# Autodesk Inventor assembly: Custom_Delta_Assembly
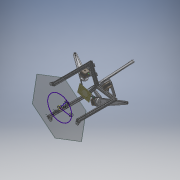
[picture p0: Inventor's stored thumbnail of the model, 180x180]
Saved by Autodesk Inventor 2019 (Build 230136000, 136)
## iProperties
Created: 2019-07-06
Part Number: Custom_Delta_Assembly
Document SubType Name: Assembly
Designer: Jorian Brusind
Author: Jorian Brusind
## Documents named in this file (15)
- C:\Users\Jorian Brusind\Documents\GitHub\ECE44x_Senior_Design\Design files\Delta Robot Arm\Inventor Files\Custom_Delta\Custom_Delta_Assembly.iam
- C:\Users\Jorian Brusind\Documents\GitHub\ECE44x_Senior_Design\Design files\Delta Robot Arm\Inventor Files\Custom_Delta\Stepper_Face.ipt
- C:\Users\Jorian Brusind\Documents\GitHub\ECE44x_Senior_Design\Design files\Delta Robot Arm\Inventor Files\nema-17-stepper-motor-with-v2-damper-1.snapshot.3\Nema 17  Stepper Motor length 34mm.ipt
- C:\Users\Jorian Brusind\Documents\GitHub\ECE44x_Senior_Design\Design files\Delta Robot Arm\Inventor Files\Stepper_Collar\products\12488\step\model.ipt
- C:\Users\Jorian Brusind\Documents\GitHub\ECE44x_Senior_Design\Design files\Delta Robot Arm\Inventor Files\Custom_Delta\Delta_Arm.ipt
- C:\Users\Jorian Brusind\Documents\GitHub\ECE44x_Senior_Design\Design files\Delta Robot Arm\Inventor Files\Custom_Delta\Delta_Top.ipt
- C:\Users\Jorian Brusind\Documents\GitHub\ECE44x_Senior_Design\Design files\Delta Robot Arm\Inventor Files\McMaster Files\59935K140_METRIC BALL JOINT ROD END.ipt
- C:\Users\Jorian Brusind\Documents\GitHub\ECE44x_Senior_Design\Design files\PetriFilm\PetriFilm.iam
- C:\Users\Jorian Brusind\Documents\GitHub\ECE44x_Senior_Design\Design files\Delta Robot Arm\Inventor Files\McMaster Files\5537T501_ALUMINUM T-SLOTTED FRAMING EXTRUSION.ipt
- C:\Users\Jorian Brusind\Documents\GitHub\ECE44x_Senior_Design\Design files\Delta Robot Arm\Inventor Files\McMaster Files\5537T518_T-SLOTTED FRAMING.ipt
- C:\Users\Jorian Brusind\Documents\GitHub\ECE44x_Senior_Design\Design files\Delta Robot Arm\Inventor Files\McMaster Files\6In_ALUMINUM T-SLOTTED FRAMING EXTRUSION.ipt
- C:\Users\Jorian Brusind\Documents\GitHub\ECE44x_Senior_Design\Design files\Delta Robot Arm\Inventor Files\McMaster Files\98861A050_LOW-STRENGTH STEEL THREADED ROD.ipt
- C:\Users\Jorian Brusind\Documents\GitHub\ECE44x_Senior_Design\Design files\Delta Robot Arm\Inventor Files\Custom_Delta\Custom_Delta_End_Effector.ipt
- C:\Users\Jorian Brusind\Documents\GitHub\ECE44x_Senior_Design\Design files\Delta Robot Arm\Inventor Files\Custom_Delta\80_20_Connector.ipt
- C:\Users\Jorian Brusind\Documents\GitHub\ECE44x_Senior_Design\Design files\Delta Robot Arm\Inventor Files\Metric bolt\Bolt M3 10mm.ipt
## Components (44 placed, 14 different names)
1. Stepper_Face:1 — Mate:1, Mate:2, Mate:3, Mate:126, Flush:20, Flush:23
2. Nema 17  Stepper Motor length 34mm:1 — Mate:1, Mate:2, Mate:3, Mate:4, Flush:1, Mate:135
3. model:1 — Mate:4, Flush:1, Mate:134, Mate:136
4. Delta_Arm:1 — Mate:134, Mate:135, Mate:136, Mate:145, Mate:146, Mate:147, Mate:148
5. Stepper_Face:2 — Mate:125, Flush:18, Flush:24
6. Nema 17  Stepper Motor length 34mm:2 — Mate:131
7. model:2 — Mate:132, Mate:133, Mate:186
8. Delta_Arm:2 — Mate:131, Mate:132, Mate:133, Mate:149, Mate:150, Mate:151, Mate:152, Mate:187
9. Stepper_Face:3 — Mate:127, Flush:21, Flush:22
10. Nema 17  Stepper Motor length 34mm:3 — Mate:128
11. model:3 — Mate:129, Mate:130
12. Delta_Arm:3 — Mate:128, Flush:17, Mate:129, Mate:130, Mate:137, Mate:138, Mate:139, Mate:140
13. Delta_Top:1 — Mate:103, Mate:105, Mate:106, Mate:107, Mate:109, Mate:110, Mate:111, Mate:112, Mate:113, Mate:114, Mate:115, Mate:116, Mate:182, Mate:185
14. 59935K140_METRIC BALL JOINT ROD END:2 — Mate:145, Mate:146, Mate:159, Mate:160
15. 59935K140_METRIC BALL JOINT ROD END:3 — Mate:151, Mate:152, Mate:153, Mate:154
16. 59935K140_METRIC BALL JOINT ROD END:5 — Mate:137, Mate:138, Mate:143, Mate:144
17. 59935K140_METRIC BALL JOINT ROD END:6 — Mate:139, Mate:140, Mate:141, Mate:142
18. 59935K140_METRIC BALL JOINT ROD END:7 — Mate:147, Mate:148, Mate:157, Mate:158
19. 59935K140_METRIC BALL JOINT ROD END:8 — Mate:149, Mate:150, Mate:155, Mate:156
20. PetriFilm:1 [sub-assembly] — Mate:181, Mate:183
21. 5537T518_T-SLOTTED FRAMING:1 — Mate:106, Mate:107, Mate:119
22. 5537T518_T-SLOTTED FRAMING:2 — Mate:103, Mate:105, Mate:118
23. 5537T518_T-SLOTTED FRAMING:3 — Mate:109, Mate:110, Mate:117
24. 6In_ALUMINUM T-SLOTTED FRAMING EXTRUSION:1 — Flush:5, Mate:121, Flush:6, Mate:126, Flush:20, Flush:23
25. 6In_ALUMINUM T-SLOTTED FRAMING EXTRUSION:2 — Flush:9, Flush:10, Mate:123, Mate:125, Flush:18, Flush:24, Mate:184
26. 6In_ALUMINUM T-SLOTTED FRAMING EXTRUSION:3 — Flush:7, Flush:8, Mate:122, Mate:127, Flush:21, Flush:22
27. 5537T501_ALUMINUM T-SLOTTED FRAMING EXTRUSION:1 — Mate:112, Mate:114, Mate:118, Flush:5, Mate:121, Flush:6
28. 5537T501_ALUMINUM T-SLOTTED FRAMING EXTRUSION:2 — Mate:111, Mate:115, Mate:119, Flush:7, Flush:8, Mate:122
29. 5537T501_ALUMINUM T-SLOTTED FRAMING EXTRUSION:3 — Mate:113, Mate:116, Mate:117, Flush:9, Flush:10, Mate:123
30. 98861A050_LOW-STRENGTH STEEL THREADED ROD:1 — Mate:143, Mate:144, Mate:163, Mate:164
31. 98861A050_LOW-STRENGTH STEEL THREADED ROD:2 — Mate:153, Mate:154, Mate:168, Mate:170
32. 98861A050_LOW-STRENGTH STEEL THREADED ROD:3 — Mate:155, Mate:156, Mate:167, Mate:169
33. 98861A050_LOW-STRENGTH STEEL THREADED ROD:4 — Mate:141, Mate:142, Mate:161, Mate:162
34. 98861A050_LOW-STRENGTH STEEL THREADED ROD:5 — Mate:157, Mate:158, Mate:165, Mate:172
35. 98861A050_LOW-STRENGTH STEEL THREADED ROD:6 — Mate:159, Mate:160, Mate:166, Mate:171
36. 59935K140_METRIC BALL JOINT ROD END:9 — Mate:165, Mate:172, Mate:174, Mate:178
37. 59935K140_METRIC BALL JOINT ROD END:10 — Mate:163, Mate:164, Mate:176
38. 59935K140_METRIC BALL JOINT ROD END:11 — Mate:166, Mate:171, Mate:174
39. 59935K140_METRIC BALL JOINT ROD END:12 — Mate:161, Mate:162, Mate:176, Mate:180
40. 59935K140_METRIC BALL JOINT ROD END:13 — Mate:168, Mate:170, Mate:175
41. 59935K140_METRIC BALL JOINT ROD END:14 — Mate:167, Mate:169, Mate:175, Mate:179
42. Custom_Delta_End_Effector:1 — Mate:178, Mate:179, Mate:180, Mate:181, Mate:182, Mate:183
43. 80_20_Connector:1 — Mate:184, Mate:185
44. Bolt M3 10mm:1 — Mate:186, Mate:187
## Relationships (107: Mate 91, Flush 16)
- Mate:1: Stepper_Face:1 ↔ Nema 17  Stepper Motor length 34mm:1
- Mate:2: Stepper_Face:1 ↔ Nema 17  Stepper Motor length 34mm:1
- Mate:3: Stepper_Face:1 ↔ Nema 17  Stepper Motor length 34mm:1
- Mate:4: Nema 17  Stepper Motor length 34mm:1 ↔ model:1
- Flush:1: Nema 17  Stepper Motor length 34mm:1 ↔ model:1
- [Mate]: Stepper_Face:2 ↔ Nema 17  Stepper Motor length 34mm:2
- [Mate]: Stepper_Face:2 ↔ Nema 17  Stepper Motor length 34mm:2
- [Mate]: Stepper_Face:2 ↔ Nema 17  Stepper Motor length 34mm:2
- [Mate]: Nema 17  Stepper Motor length 34mm:2 ↔ model:2
- [Flush]: Nema 17  Stepper Motor length 34mm:2 ↔ model:2
- [Mate]: Stepper_Face:3 ↔ Nema 17  Stepper Motor length 34mm:3
- [Mate]: Stepper_Face:3 ↔ Nema 17  Stepper Motor length 34mm:3
- [Mate]: Stepper_Face:3 ↔ Nema 17  Stepper Motor length 34mm:3
- [Mate]: Nema 17  Stepper Motor length 34mm:3 ↔ model:3
- [Flush]: Nema 17  Stepper Motor length 34mm:3 ↔ model:3
- Mate:103: Delta_Top:1 ↔ 5537T518_T-SLOTTED FRAMING:2
- Mate:105: Delta_Top:1 ↔ 5537T518_T-SLOTTED FRAMING:2
- Mate:106: Delta_Top:1 ↔ 5537T518_T-SLOTTED FRAMING:1
- Mate:107: Delta_Top:1 ↔ 5537T518_T-SLOTTED FRAMING:1
- Mate:109: Delta_Top:1 ↔ 5537T518_T-SLOTTED FRAMING:3
- Mate:110: Delta_Top:1 ↔ 5537T518_T-SLOTTED FRAMING:3
- Mate:111: Delta_Top:1 ↔ 5537T501_ALUMINUM T-SLOTTED FRAMING EXTRUSION:2
- Mate:112: Delta_Top:1 ↔ 5537T501_ALUMINUM T-SLOTTED FRAMING EXTRUSION:1
- Mate:113: Delta_Top:1 ↔ 5537T501_ALUMINUM T-SLOTTED FRAMING EXTRUSION:3
- Mate:114: Delta_Top:1 ↔ 5537T501_ALUMINUM T-SLOTTED FRAMING EXTRUSION:1
- Mate:115: Delta_Top:1 ↔ 5537T501_ALUMINUM T-SLOTTED FRAMING EXTRUSION:2
- Mate:116: Delta_Top:1 ↔ 5537T501_ALUMINUM T-SLOTTED FRAMING EXTRUSION:3
- Mate:117: 5537T518_T-SLOTTED FRAMING:3 ↔ 5537T501_ALUMINUM T-SLOTTED FRAMING EXTRUSION:3
- Mate:118: 5537T518_T-SLOTTED FRAMING:2 ↔ 5537T501_ALUMINUM T-SLOTTED FRAMING EXTRUSION:1
- Mate:119: 5537T518_T-SLOTTED FRAMING:1 ↔ 5537T501_ALUMINUM T-SLOTTED FRAMING EXTRUSION:2
- Flush:5: 6In_ALUMINUM T-SLOTTED FRAMING EXTRUSION:1 ↔ 5537T501_ALUMINUM T-SLOTTED FRAMING EXTRUSION:1
- Mate:121: 6In_ALUMINUM T-SLOTTED FRAMING EXTRUSION:1 ↔ 5537T501_ALUMINUM T-SLOTTED FRAMING EXTRUSION:1
- Flush:6: 6In_ALUMINUM T-SLOTTED FRAMING EXTRUSION:1 ↔ 5537T501_ALUMINUM T-SLOTTED FRAMING EXTRUSION:1
- Flush:7: 6In_ALUMINUM T-SLOTTED FRAMING EXTRUSION:3 ↔ 5537T501_ALUMINUM T-SLOTTED FRAMING EXTRUSION:2
- Flush:8: 6In_ALUMINUM T-SLOTTED FRAMING EXTRUSION:3 ↔ 5537T501_ALUMINUM T-SLOTTED FRAMING EXTRUSION:2
- Mate:122: 6In_ALUMINUM T-SLOTTED FRAMING EXTRUSION:3 ↔ 5537T501_ALUMINUM T-SLOTTED FRAMING EXTRUSION:2
- Flush:9: 6In_ALUMINUM T-SLOTTED FRAMING EXTRUSION:2 ↔ 5537T501_ALUMINUM T-SLOTTED FRAMING EXTRUSION:3
- Flush:10: 6In_ALUMINUM T-SLOTTED FRAMING EXTRUSION:2 ↔ 5537T501_ALUMINUM T-SLOTTED FRAMING EXTRUSION:3
- Mate:123: 6In_ALUMINUM T-SLOTTED FRAMING EXTRUSION:2 ↔ 5537T501_ALUMINUM T-SLOTTED FRAMING EXTRUSION:3
- Mate:125: Stepper_Face:2 ↔ 6In_ALUMINUM T-SLOTTED FRAMING EXTRUSION:2
- Mate:126: Stepper_Face:1 ↔ 6In_ALUMINUM T-SLOTTED FRAMING EXTRUSION:1
- Mate:127: Stepper_Face:3 ↔ 6In_ALUMINUM T-SLOTTED FRAMING EXTRUSION:3
- Mate:128: Nema 17  Stepper Motor length 34mm:3 ↔ Delta_Arm:3
- Flush:17: Delta_Arm:3
- Mate:129: model:3 ↔ Delta_Arm:3
- Mate:130: model:3 ↔ Delta_Arm:3
- Mate:131: Nema 17  Stepper Motor length 34mm:2 ↔ Delta_Arm:2
- Mate:132: model:2 ↔ Delta_Arm:2
- Mate:133: model:2 ↔ Delta_Arm:2
- Mate:134: model:1 ↔ Delta_Arm:1
- Mate:135: Nema 17  Stepper Motor length 34mm:1 ↔ Delta_Arm:1
- Mate:136: model:1 ↔ Delta_Arm:1
- Mate:137: Delta_Arm:3 ↔ 59935K140_METRIC BALL JOINT ROD END:5
- Mate:138: Delta_Arm:3 ↔ 59935K140_METRIC BALL JOINT ROD END:5
- Mate:139: Delta_Arm:3 ↔ 59935K140_METRIC BALL JOINT ROD END:6
- Mate:140: Delta_Arm:3 ↔ 59935K140_METRIC BALL JOINT ROD END:6
- Mate:141: 59935K140_METRIC BALL JOINT ROD END:6 ↔ 98861A050_LOW-STRENGTH STEEL THREADED ROD:4
- Mate:142: 59935K140_METRIC BALL JOINT ROD END:6 ↔ 98861A050_LOW-STRENGTH STEEL THREADED ROD:4
- Mate:143: 59935K140_METRIC BALL JOINT ROD END:5 ↔ 98861A050_LOW-STRENGTH STEEL THREADED ROD:1
- Mate:144: 59935K140_METRIC BALL JOINT ROD END:5 ↔ 98861A050_LOW-STRENGTH STEEL THREADED ROD:1
- Mate:145: Delta_Arm:1 ↔ 59935K140_METRIC BALL JOINT ROD END:2
- Mate:146: Delta_Arm:1 ↔ 59935K140_METRIC BALL JOINT ROD END:2
- Mate:147: Delta_Arm:1 ↔ 59935K140_METRIC BALL JOINT ROD END:7
- Mate:148: Delta_Arm:1 ↔ 59935K140_METRIC BALL JOINT ROD END:7
- Mate:149: Delta_Arm:2 ↔ 59935K140_METRIC BALL JOINT ROD END:8
- Mate:150: Delta_Arm:2 ↔ 59935K140_METRIC BALL JOINT ROD END:8
- Mate:151: Delta_Arm:2 ↔ 59935K140_METRIC BALL JOINT ROD END:3
- Mate:152: Delta_Arm:2 ↔ 59935K140_METRIC BALL JOINT ROD END:3
- Mate:153: 59935K140_METRIC BALL JOINT ROD END:3 ↔ 98861A050_LOW-STRENGTH STEEL THREADED ROD:2
- Mate:154: 59935K140_METRIC BALL JOINT ROD END:3 ↔ 98861A050_LOW-STRENGTH STEEL THREADED ROD:2
- Mate:155: 59935K140_METRIC BALL JOINT ROD END:8 ↔ 98861A050_LOW-STRENGTH STEEL THREADED ROD:3
- Mate:156: 59935K140_METRIC BALL JOINT ROD END:8 ↔ 98861A050_LOW-STRENGTH STEEL THREADED ROD:3
- Mate:157: 59935K140_METRIC BALL JOINT ROD END:7 ↔ 98861A050_LOW-STRENGTH STEEL THREADED ROD:5
- Mate:158: 59935K140_METRIC BALL JOINT ROD END:7 ↔ 98861A050_LOW-STRENGTH STEEL THREADED ROD:5
- Mate:159: 59935K140_METRIC BALL JOINT ROD END:2 ↔ 98861A050_LOW-STRENGTH STEEL THREADED ROD:6
- Mate:160: 59935K140_METRIC BALL JOINT ROD END:2 ↔ 98861A050_LOW-STRENGTH STEEL THREADED ROD:6
- Mate:161: 98861A050_LOW-STRENGTH STEEL THREADED ROD:4 ↔ 59935K140_METRIC BALL JOINT ROD END:12
- Mate:162: 98861A050_LOW-STRENGTH STEEL THREADED ROD:4 ↔ 59935K140_METRIC BALL JOINT ROD END:12
- Mate:163: 98861A050_LOW-STRENGTH STEEL THREADED ROD:1 ↔ 59935K140_METRIC BALL JOINT ROD END:10
- Mate:164: 98861A050_LOW-STRENGTH STEEL THREADED ROD:1 ↔ 59935K140_METRIC BALL JOINT ROD END:10
- Mate:165: 98861A050_LOW-STRENGTH STEEL THREADED ROD:5 ↔ 59935K140_METRIC BALL JOINT ROD END:9
- Mate:166: 98861A050_LOW-STRENGTH STEEL THREADED ROD:6 ↔ 59935K140_METRIC BALL JOINT ROD END:11
- Mate:167: 98861A050_LOW-STRENGTH STEEL THREADED ROD:3 ↔ 59935K140_METRIC BALL JOINT ROD END:14
- Mate:168: 98861A050_LOW-STRENGTH STEEL THREADED ROD:2 ↔ 59935K140_METRIC BALL JOINT ROD END:13
- Mate:169: 98861A050_LOW-STRENGTH STEEL THREADED ROD:3 ↔ 59935K140_METRIC BALL JOINT ROD END:14
- Mate:170: 98861A050_LOW-STRENGTH STEEL THREADED ROD:2 ↔ 59935K140_METRIC BALL JOINT ROD END:13
- Mate:171: 98861A050_LOW-STRENGTH STEEL THREADED ROD:6 ↔ 59935K140_METRIC BALL JOINT ROD END:11
- Mate:172: 98861A050_LOW-STRENGTH STEEL THREADED ROD:5 ↔ 59935K140_METRIC BALL JOINT ROD END:9
- Mate:174: 59935K140_METRIC BALL JOINT ROD END:9 ↔ 59935K140_METRIC BALL JOINT ROD END:11
- Mate:175: 59935K140_METRIC BALL JOINT ROD END:13 ↔ 59935K140_METRIC BALL JOINT ROD END:14
- Mate:176: 59935K140_METRIC BALL JOINT ROD END:10 ↔ 59935K140_METRIC BALL JOINT ROD END:12
- Flush:18: Stepper_Face:2 ↔ 6In_ALUMINUM T-SLOTTED FRAMING EXTRUSION:2
- Flush:20: Stepper_Face:1 ↔ 6In_ALUMINUM T-SLOTTED FRAMING EXTRUSION:1
- Flush:21: Stepper_Face:3 ↔ 6In_ALUMINUM T-SLOTTED FRAMING EXTRUSION:3
- Flush:22 (112.406 mm): Stepper_Face:3 ↔ 6In_ALUMINUM T-SLOTTED FRAMING EXTRUSION:3
- Flush:23 (112.206 mm): Stepper_Face:1 ↔ 6In_ALUMINUM T-SLOTTED FRAMING EXTRUSION:1
- Flush:24 (112.406 mm): Stepper_Face:2 ↔ 6In_ALUMINUM T-SLOTTED FRAMING EXTRUSION:2
- Mate:178: 59935K140_METRIC BALL JOINT ROD END:9 ↔ Custom_Delta_End_Effector:1
- Mate:179: 59935K140_METRIC BALL JOINT ROD END:14 ↔ Custom_Delta_End_Effector:1
- Mate:180: 59935K140_METRIC BALL JOINT ROD END:12 ↔ Custom_Delta_End_Effector:1
- Mate:181: PetriFilm:1 ↔ Custom_Delta_End_Effector:1
- Mate:182: Delta_Top:1 ↔ Custom_Delta_End_Effector:1
- Mate:183 (-25 mm): PetriFilm:1 ↔ Custom_Delta_End_Effector:1
- Mate:184: 6In_ALUMINUM T-SLOTTED FRAMING EXTRUSION:2 ↔ 80_20_Connector:1
- Mate:185: Delta_Top:1 ↔ 80_20_Connector:1
- Mate:186: model:2 ↔ Bolt M3 10mm:1
- Mate:187: Delta_Arm:2 ↔ Bolt M3 10mm:1
## Named parameters: d14_d5 = 0 mm, d17_d0 = 0 mm, d18_d1 = 0 mm, d19_d2 = 0 mm, d20_d3 = 0 mm, d22_d5 = 0 mm, d25_d0 = 0 mm, d26_d1 = 0 mm, d27_d2 = 0 mm, d28_d3 = 0 mm
